# Autodesk Inventor assembly: Undercarriage
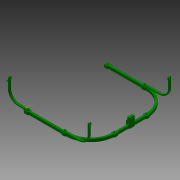
[picture p0: Inventor's stored thumbnail of the model, 180x180]
Saved by Autodesk Inventor 2014 SP1 (Build 180222100, 222)
## iProperties
Created: 2017-01-18
Part Number: Undercarriage
Document SubType Name: Assembly
Designer: danielsikar
Author: danielsikar
## Documents named in this file (6)
- C:\Users\danielsikar\Documents\Inventor\IoT-Trike\Assemblies\Undercarriage.iam
- C:\Users\danielsikar\Documents\Inventor\IoT-Trike\Parts\UndercarriageLeft.ipt
- C:\Users\danielsikar\Documents\Inventor\IoT-Trike\Parts\UndercarriageRight.ipt
- C:\Users\danielsikar\Documents\Inventor\IoT-Trike\Parts\BackNetHookLeft.ipt
- C:\Users\danielsikar\Documents\Inventor\IoT-Trike\Parts\FrontNetHook.ipt
- C:\Users\danielsikar\Documents\Inventor\IoT-Trike\Parts\FrontNetHookLeft.ipt
## Components (5 placed, 5 different names)
1. UndercarriageLeft:1 — Mate:1, Mate:2, Mate:5, Mate:6, Mate:7, Mate:8
2. UndercarriageRight:1 — Mate:3, Mate:4, Mate:6, Mate:9, Flush:1, Mate:10
3. BackNetHookLeft:1 — Mate:7, Mate:8
4. FrontNetHook:1 — Mate:9, Flush:2, Mate:10
5. FrontNetHookLeft:1 — Flush:4
## Relationships (14: Mate 10, Flush 4)
- Mate:1: UndercarriageLeft:1
- Mate:2: UndercarriageLeft:1
- Mate:3: UndercarriageRight:1
- Mate:4: UndercarriageRight:1
- Mate:5: UndercarriageLeft:1
- Mate:6: UndercarriageLeft:1 ↔ UndercarriageRight:1
- Mate:7: UndercarriageLeft:1 ↔ BackNetHookLeft:1
- Mate:8: UndercarriageLeft:1 ↔ BackNetHookLeft:1
- Mate:9: UndercarriageRight:1 ↔ FrontNetHook:1
- Flush:1 (1 mm): UndercarriageRight:1
- Flush:2: FrontNetHook:1
- Mate:10: UndercarriageRight:1 ↔ FrontNetHook:1
- Flush:3 (125.5 mm)
- Flush:4: FrontNetHookLeft:1
